# Autodesk Inventor assembly: testframe
(part 2 of 2)
- Mate:428: STRU_018_AngleBracket_62:3 ↔ COTS_95615A120_Medium-Strength Steel Nylon-Insert Locknut:36
- Mate:429: STRU_018_AngleBracket_62:3 ↔ COTS_95615A120_Medium-Strength Steel Nylon-Insert Locknut:33
- Mate:430: STRU_018_AngleBracket_62:3 ↔ COTS_95615A120_Medium-Strength Steel Nylon-Insert Locknut:31
- Mate:431: STRU_018_AngleBracket_62:3 ↔ COTS_95615A120_Medium-Strength Steel Nylon-Insert Locknut:35
- Mate:432: COTS_91251A539_Black-Oxide Alloy Steel Socket Head Screw (1):2 ↔ COTS_95462A029_Medium-Strength Steel Hex Nut (2):1
- Mate:433: COTS_91251A539_Black-Oxide Alloy Steel Socket Head Screw (1):2 ↔ STRU_019_RubberWasher:1
- Mate:434: STRU_017_AngleBracket_90_Plastic:2 ↔ STRU_019_RubberWasher:1
- Mate:435: STRU_017_AngleBracket_90_Plastic:2 ↔ STRU_019_RubberWasher:1
- Mate:436: COTS_95462A029_Medium-Strength Steel Hex Nut (2):1 ↔ STRU_019_RubberWasher:1
- [Mate]: COTS_95462A029_Medium-Strength Steel Hex Nut (2):2 ↔ STRU_019_RubberWasher:2
- Mate:438: COTS_95462A029_Medium-Strength Steel Hex Nut (2):2 ↔ STRU_019_RubberWasher:2
- Mate:439: COTS_91251A539_Black-Oxide Alloy Steel Socket Head Screw (1):1 ↔ COTS_95462A029_Medium-Strength Steel Hex Nut (2):2
- Flush:59: STRU_019_RubberWasher:1 ↔ STRU_019_RubberWasher:2
- Mate:440: STRU_017_AngleBracket_90_Plastic:2 ↔ STRU_019_RubberWasher:2
- [Mate]: COTS_95462A029_Medium-Strength Steel Hex Nut (2):3 ↔ STRU_019_RubberWasher:3
- Mate:442: COTS_90044A123_Black-Oxide Alloy Steel Socket Head Screw:30 ↔ COTS_95462A029_Medium-Strength Steel Hex Nut (2):3
- Mate:443: COTS_90044A123_Black-Oxide Alloy Steel Socket Head Screw:30 ↔ STRU_019_RubberWasher:3
- Mate:444: STRU_017_AngleBracket_90_Plastic:2 ↔ STRU_019_RubberWasher:3
- Mate:445: STRU_017_AngleBracket_90_Plastic:2 ↔ STRU_019_RubberWasher:3
- [Mate]: COTS_95462A029_Medium-Strength Steel Hex Nut (2):4 ↔ STRU_019_RubberWasher:4
- Mate:447: COTS_95462A029_Medium-Strength Steel Hex Nut (2):4 ↔ STRU_019_RubberWasher:4
- Mate:448: COTS_90044A123_Black-Oxide Alloy Steel Socket Head Screw:29 ↔ COTS_95462A029_Medium-Strength Steel Hex Nut (2):4
- Mate:449: STRU_017_AngleBracket_90_Plastic:2 ↔ STRU_019_RubberWasher:4
- Flush:60: STRU_019_RubberWasher:3 ↔ STRU_019_RubberWasher:4
- [Mate]: COTS_95462A029_Medium-Strength Steel Hex Nut (2):5 ↔ STRU_019_RubberWasher:5
- [Mate]: COTS_95462A029_Medium-Strength Steel Hex Nut (2):5 ↔ STRU_019_RubberWasher:5
- Mate:452: COTS_91251A539_Black-Oxide Alloy Steel Socket Head Screw (1):5 ↔ COTS_95462A029_Medium-Strength Steel Hex Nut (2):5
- Mate:453: STRU_017_AngleBracket_90_Plastic:1 ↔ STRU_019_RubberWasher:5
- Mate:454: STRU_017_AngleBracket_90_Plastic:1 ↔ STRU_019_RubberWasher:5
- [Mate]: COTS_95462A029_Medium-Strength Steel Hex Nut (2):6 ↔ STRU_019_RubberWasher:6
- [Mate]: COTS_95462A029_Medium-Strength Steel Hex Nut (2):6 ↔ STRU_019_RubberWasher:6
- Mate:457: COTS_91251A539_Black-Oxide Alloy Steel Socket Head Screw (1):4 ↔ COTS_95462A029_Medium-Strength Steel Hex Nut (2):6
- Mate:458: STRU_017_AngleBracket_90_Plastic:1 ↔ STRU_019_RubberWasher:6
- Flush:61: STRU_019_RubberWasher:5 ↔ STRU_019_RubberWasher:6
- [Mate]: COTS_95462A029_Medium-Strength Steel Hex Nut (2):7 ↔ STRU_019_RubberWasher:7
- [Mate]: COTS_95462A029_Medium-Strength Steel Hex Nut (2):7 ↔ STRU_019_RubberWasher:7
- Mate:461: COTS_90044A123_Black-Oxide Alloy Steel Socket Head Screw:27 ↔ COTS_95462A029_Medium-Strength Steel Hex Nut (2):7
- Mate:462: STRU_017_AngleBracket_90_Plastic:1 ↔ STRU_019_RubberWasher:7
- Mate:463: STRU_017_AngleBracket_90_Plastic:1 ↔ STRU_019_RubberWasher:7
- [Mate]: COTS_95462A029_Medium-Strength Steel Hex Nut (2):8 ↔ STRU_019_RubberWasher:8
- [Mate]: COTS_95462A029_Medium-Strength Steel Hex Nut (2):8 ↔ STRU_019_RubberWasher:8
- Mate:466: COTS_90044A123_Black-Oxide Alloy Steel Socket Head Screw:28 ↔ COTS_95462A029_Medium-Strength Steel Hex Nut (2):8
- Mate:467: STRU_017_AngleBracket_90_Plastic:1 ↔ STRU_019_RubberWasher:8
- Flush:62: STRU_019_RubberWasher:7 ↔ STRU_019_RubberWasher:8
- Mate:470: STRU_002_BilletPole_20.56in_Angled:1 ↔ STRU_001_BilletBlock:22
- Mate:471: STRU_002_BilletPole_20.56in_Angled:1 ↔ STRU_001_BilletBlock:22
- Mate:472: STRU_023_Kenji_11in:1 ↔ STRU_001_BilletBlock:22
- Mate:473: STRU_023_Kenji_11in:1 ↔ STRU_001_BilletBlock:22
- Flush:63: STRU_002_BilletPole_20.56in_Angled:1 ↔ STRU_023_Kenji_11in:1
- Mate:475: STRU_006_BilletPole_SwerveOffset:2 ↔ STRU_023_Kenji_11in:1
- Mate:477: STRU_002_BilletPole_20.56in_Angled:2 ↔ STRU_001_BilletBlock:23
- Mate:478: STRU_002_BilletPole_20.56in_Angled:2 ↔ STRU_001_BilletBlock:23
- Mate:484: STRU_003_BilletPole_28in_Angled:2 ↔ STRU_024_BilletBlock2:1
- Mate:485: STRU_003_BilletPole_28in_Angled:2 ↔ STRU_024_BilletBlock2:6
- Mate:486: STRU_003_BilletPole_28in_Angled:2 ↔ STRU_024_BilletBlock2:5
- Mate:487: STRU_006_BilletPole_SwerveOffset:1 ↔ STRU_024_BilletBlock2:2
- Mate:488: STRU_006_BilletPole_SwerveOffset:2 ↔ STRU_024_BilletBlock2:3
- Mate:489: STRU_006_BilletPole_SwerveOffset:1 ↔ STRU_024_BilletBlock2:4
- Mate:490: STRU_003_BilletPole_28in_Angled:2 ↔ STRU_024_BilletBlock2:1
- Flush:65: STRU_001_BilletBlock:5 ↔ STRU_024_BilletBlock2:1
- Flush:66: STRU_001_BilletBlock:12 ↔ STRU_024_BilletBlock2:6
- Flush:67: STRU_024_BilletBlock2:5 ↔ STRU_024_BilletBlock2:6
- Flush:68: STRU_003_BilletPole_28in_Angled:2 ↔ STRU_003_BilletPole_28in_Angled_Unique:1
- Flush:69: STRU_024_BilletBlock2:2 ↔ STRU_024_BilletBlock2:5
- Mate:491: STRU_003_BilletPole_28in_Angled:2 ↔ STRU_024_BilletBlock2:5
- Mate:492: STRU_003_BilletPole_28in_Angled:2 ↔ STRU_024_BilletBlock2:2
- Mate:493: STRU_003_BilletPole_28in_Angled:2 ↔ STRU_024_BilletBlock2:6
- Mate:494: STRU_006_BilletPole_SwerveOffset:1 ↔ STRU_024_BilletBlock2:4
- Mate:495: STRU_006_BilletPole_SwerveOffset:2 ↔ STRU_024_BilletBlock2:3
- Flush:70: STRU_024_BilletBlock2:3 ↔ STRU_024_BilletBlock2:4
- Mate:497: STRU_009_FrameBracket_90:1 ↔ COTS_90357A021_Ultra-Low-Profile Socket Head Screw:1
- Mate:498: STRU_009_FrameBracket_90:1 ↔ COTS_90357A021_Ultra-Low-Profile Socket Head Screw:1
- Mate:499: STRU_009_FrameBracket_90:1 ↔ COTS_90357A018_Ultra-Low-Profile Socket Head Screw:1
- Mate:500: STRU_009_FrameBracket_90:1 ↔ COTS_90357A018_Ultra-Low-Profile Socket Head Screw:1
- Mate:501: STRU_009_FrameBracket_90:1 ↔ COTS_90357A018_Ultra-Low-Profile Socket Head Screw:2
- Mate:502: STRU_009_FrameBracket_90:1 ↔ COTS_90357A018_Ultra-Low-Profile Socket Head Screw:3
- Mate:503: STRU_009_FrameBracket_90:1 ↔ COTS_90357A018_Ultra-Low-Profile Socket Head Screw:4
- Mate:504: STRU_009_FrameBracket_90:4 ↔ COTS_90357A018_Ultra-Low-Profile Socket Head Screw:5
- Mate:505: STRU_009_FrameBracket_90:4 ↔ COTS_90357A018_Ultra-Low-Profile Socket Head Screw:6
- Mate:506: STRU_009_FrameBracket_90:4 ↔ COTS_90357A018_Ultra-Low-Profile Socket Head Screw:7
- Mate:507: STRU_009_FrameBracket_90:4 ↔ COTS_90357A018_Ultra-Low-Profile Socket Head Screw:8
- Mate:508: STRU_009_FrameBracket_90:4 ↔ COTS_90357A018_Ultra-Low-Profile Socket Head Screw:5
- Mate:509: STRU_009_FrameBracket_90:4 ↔ COTS_90357A018_Ultra-Low-Profile Socket Head Screw:6
- Mate:510: STRU_009_FrameBracket_90:4 ↔ COTS_90357A018_Ultra-Low-Profile Socket Head Screw:7
- Mate:511: STRU_009_FrameBracket_90:4 ↔ COTS_90357A018_Ultra-Low-Profile Socket Head Screw:8
- Mate:512: COTS_95615A120_Medium-Strength Steel Nylon-Insert Locknut:12 ↔ COTS_90357A018_Ultra-Low-Profile Socket Head Screw:8
- Mate:513: COTS_95615A120_Medium-Strength Steel Nylon-Insert Locknut:11 ↔ COTS_90357A018_Ultra-Low-Profile Socket Head Screw:7
- Mate:514: COTS_95615A120_Medium-Strength Steel Nylon-Insert Locknut:9 ↔ COTS_90357A018_Ultra-Low-Profile Socket Head Screw:5
- Mate:515: COTS_95615A120_Medium-Strength Steel Nylon-Insert Locknut:10 ↔ COTS_90357A018_Ultra-Low-Profile Socket Head Screw:6
- Mate:516: STRU_009_FrameBracket_90:1 ↔ COTS_90357A018_Ultra-Low-Profile Socket Head Screw:2
- Mate:517: STRU_009_FrameBracket_90:1 ↔ COTS_90357A018_Ultra-Low-Profile Socket Head Screw:4
- Mate:518: STRU_009_FrameBracket_90:1 ↔ COTS_90357A018_Ultra-Low-Profile Socket Head Screw:3
- Mate:519: COTS_95615A120_Medium-Strength Steel Nylon-Insert Locknut:3 ↔ COTS_90357A018_Ultra-Low-Profile Socket Head Screw:3
- Mate:520: COTS_95615A120_Medium-Strength Steel Nylon-Insert Locknut:4 ↔ COTS_90357A018_Ultra-Low-Profile Socket Head Screw:4
- Mate:521: COTS_95615A120_Medium-Strength Steel Nylon-Insert Locknut:2 ↔ COTS_90357A018_Ultra-Low-Profile Socket Head Screw:1
- Mate:522: COTS_95615A120_Medium-Strength Steel Nylon-Insert Locknut:1 ↔ COTS_90357A018_Ultra-Low-Profile Socket Head Screw:2
- Mate:523: STRU_009_FrameBracket_90:4 ↔ COTS_90357A021_Ultra-Low-Profile Socket Head Screw:2
- Mate:524: STRU_009_FrameBracket_90:4 ↔ COTS_90357A021_Ultra-Low-Profile Socket Head Screw:2
- Mate:525: STRU_006_BilletPole_SwerveOffset:2 ↔ COTS_91251A352_Black-Oxide Alloy Steel Socket Head:1
- Mate:526: STRU_006_BilletPole_SwerveOffset:2 ↔ COTS_91251A352_Black-Oxide Alloy Steel Socket Head:1
- Mate:527: STRU_002_BilletPole_20.56in_Angled:1 ↔ COTS_91251A352_Black-Oxide Alloy Steel Socket Head:2
- Mate:528: STRU_002_BilletPole_20.56in_Angled:1 ↔ COTS_91251A352_Black-Oxide Alloy Steel Socket Head:2
- Mate:529: STRU_006_BilletPole_SwerveOffset:1 ↔ COTS_91251A352_Black-Oxide Alloy Steel Socket Head:3
- Mate:530: STRU_006_BilletPole_SwerveOffset:1 ↔ COTS_91251A352_Black-Oxide Alloy Steel Socket Head:3
- Mate:531: STRU_002_BilletPole_20.56in_Angled:2 ↔ COTS_91251A352_Black-Oxide Alloy Steel Socket Head:4
- Mate:532: STRU_002_BilletPole_20.56in_Angled:2 ↔ COTS_91251A352_Black-Oxide Alloy Steel Socket Head:4
- Mate:533: STRU_006_BilletPole_SwerveOffset:1 ↔ STRU_023_Kenji_11in:2
- Flush:71: STRU_002_BilletPole_20.56in_Angled:2 ↔ STRU_023_Kenji_11in:2
- Mate:534: STRU_023_Kenji_11in:2 ↔ STRU_001_BilletBlock:23
- Mate:537: STRU_007_BilletPole_11in:1 ↔ STRU_024_BilletBlock2:1
- Mate:539: STRU_024_BilletBlock2:5 ↔ STRU_026_Bryan_11in:2
- Mate:540: STRU_024_BilletBlock2:5 ↔ STRU_026_Bryan_11in:2
- Mate:541: STRU_003_BilletPole_28in_Angled:2 ↔ STRU_026_Bryan_11in:2
- Flush:73: STRU_003_BilletPole_28in_Angled:2 ↔ STRU_026_Bryan_11in:2
- Mate:542: STRU_003_BilletPole_28in_Angled:2 ↔ COTS_90357A021_Ultra-Low-Profile Socket Head Screw:3
- Mate:543: STRU_003_BilletPole_28in_Angled:2 ↔ COTS_90357A021_Ultra-Low-Profile Socket Head Screw:3
- Mate:544: STRU_003_BilletPole_28in_Angled:2 ↔ COTS_90357A021_Ultra-Low-Profile Socket Head Screw:4
- Mate:545: STRU_003_BilletPole_28in_Angled:2 ↔ COTS_90357A021_Ultra-Low-Profile Socket Head Screw:4
- Mate:546: STRU_024_BilletBlock2:6 ↔ STRU_026_Bryan_11in:3
- Mate:547: STRU_024_BilletBlock2:6 ↔ STRU_026_Bryan_11in:3
- Flush:74: STRU_003_BilletPole_28in_Angled:2 ↔ STRU_026_Bryan_11in:3
- Mate:548: STRU_003_BilletPole_28in_Angled:2 ↔ STRU_026_Bryan_11in:3
## Named parameters: d22_d7 = 0 mm, d23_d8 = 0 mm, d24_d9 = 0 mm, d25_d10 = 0 mm, d26_d11 = 0 mm, d27_d12 = 0 mm, d389_d130 = 0 mm, d393_d130 = 0 mm, d397_d130 = 0 mm, d401_d130 = 0 mm, d405_d130 = 0 mm, d409_d130 = 0 mm, d413_d130 = 0 mm, d417_d130 = 0 mm, sa_0 = 981, sa_1 = 11120.6, sa_2 = 11120.6, sa_3 = 11120.6, sa_4 = 11120.6, d560_d559 = 0 mm, d565_d559 = 0 mm, d570_d559 = 0 mm, d575_d570_d559 = 0 mm, d576_d571 = 0 mm, d580_d575_d570_d559 = 0 mm, d581_d576_d571 = 0 mm, d585_d575_d570_d559 = 0 mm, d586_d576_d571 = 0 mm, d590_d575_d570_d559 = 0 mm, d591_d576_d571 = 0 mm
note: some values were not read from the file. Shown as the stored number, unit unknown: "sa_0", "sa_1", "sa_2", "sa_3", "sa_4".
